# Autodesk Inventor assembly: mount assem
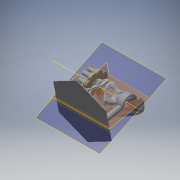
[picture p0: Inventor's stored thumbnail of the model, 180x180]
Saved by Autodesk Inventor 2019 (Build 230136000, 136)
## iProperties
Created: 2018-10-05
Part Number: mount assem
Document SubType Name: Assembly
Designer: HIVE
Author: HIVE
## Documents named in this file (8)
- E:\hive\projects\pocketpelvis\models\mounts\femur\mount assem.iam
- E:\hive\projects\pocketpelvis\models\mounts\Imported Components\pelvis_scaled1point6\pelvis_scaled1point6.ipt
- E:\hive\projects\pocketpelvis\models\mounts\femur\3945K300_HIGH-PULL RARE EARTH MAGNETIC BALL.ipt
- E:\hive\projects\pocketpelvis\models\mounts\femur\94695A250_TYPE 316 STAINLESS STEEL COUNTERSUNK WASHER.ipt
- E:\hive\projects\pocketpelvis\models\mounts\femur\mounter.ipt
- E:\hive\projects\pocketpelvis\models\mounts\femur\washer connector.ipt
- E:\hive\projects\pocketpelvis\models\mounts\femur\create hole in pelvis.ipt
- E:\hive\projects\pocketpelvis\models\mounts\femur\create rotation hole in pelvis.ipt
## Components (9 placed, 7 different names)
1. pelvis_scaled1point6:1
2. 3945K300_HIGH-PULL RARE EARTH MAGNETIC BALL:1 — Mate:3, Mate:7, Tangent:1, Mate:9
3. 3945K300_HIGH-PULL RARE EARTH MAGNETIC BALL:2 — Mate:4, Tangent:2
4. 94695A250_TYPE 316 STAINLESS STEEL COUNTERSUNK WASHER:1 — Tangent:2, Mate:11, Angle:3, Flush:2
5. 94695A250_TYPE 316 STAINLESS STEEL COUNTERSUNK WASHER:2 — Tangent:1, Mate:9, Angle:2, Tangent:3, Tangent:4, Flush:1
6. mounter:1 — Mate:7, Mate:8, Mate:10, Tangent:3, Tangent:4, Flush:3, Flush:4, Flush:5, Flush:6
7. washer connector:1 — Flush:1, Flush:2
8. create hole in pelvis:1 — Flush:3, Flush:4
9. create rotation hole in pelvis:1 — Flush:5, Flush:6
## Relationships (22: Mate 9, Flush 6, Tangent 4, Angle 3)
- Mate:3: 3945K300_HIGH-PULL RARE EARTH MAGNETIC BALL:1
- Mate:4: 3945K300_HIGH-PULL RARE EARTH MAGNETIC BALL:2
- Mate:5
- Mate:6
- Mate:7: 3945K300_HIGH-PULL RARE EARTH MAGNETIC BALL:1 ↔ mounter:1
- Mate:8: mounter:1
- Tangent:1: 3945K300_HIGH-PULL RARE EARTH MAGNETIC BALL:1 ↔ 94695A250_TYPE 316 STAINLESS STEEL COUNTERSUNK WASHER:2
- Mate:9: 3945K300_HIGH-PULL RARE EARTH MAGNETIC BALL:1 ↔ 94695A250_TYPE 316 STAINLESS STEEL COUNTERSUNK WASHER:2
- Mate:10: mounter:1
- Angle:1 (-155 deg)
- Angle:2 (0 deg): 94695A250_TYPE 316 STAINLESS STEEL COUNTERSUNK WASHER:2
- Tangent:2: 3945K300_HIGH-PULL RARE EARTH MAGNETIC BALL:2 ↔ 94695A250_TYPE 316 STAINLESS STEEL COUNTERSUNK WASHER:1
- Mate:11: 94695A250_TYPE 316 STAINLESS STEEL COUNTERSUNK WASHER:1
- Angle:3 (0 deg): 94695A250_TYPE 316 STAINLESS STEEL COUNTERSUNK WASHER:1
- Tangent:3: 94695A250_TYPE 316 STAINLESS STEEL COUNTERSUNK WASHER:2 ↔ mounter:1
- Tangent:4: 94695A250_TYPE 316 STAINLESS STEEL COUNTERSUNK WASHER:2 ↔ mounter:1
- Flush:1: 94695A250_TYPE 316 STAINLESS STEEL COUNTERSUNK WASHER:2 ↔ washer connector:1
- Flush:2: 94695A250_TYPE 316 STAINLESS STEEL COUNTERSUNK WASHER:1 ↔ washer connector:1
- Flush:3: mounter:1 ↔ create hole in pelvis:1
- Flush:4: mounter:1 ↔ create hole in pelvis:1
- Flush:5: mounter:1 ↔ create rotation hole in pelvis:1
- Flush:6: mounter:1 ↔ create rotation hole in pelvis:1
